# Autodesk Inventor assembly: ASY GBK 3310 central wall shield 7
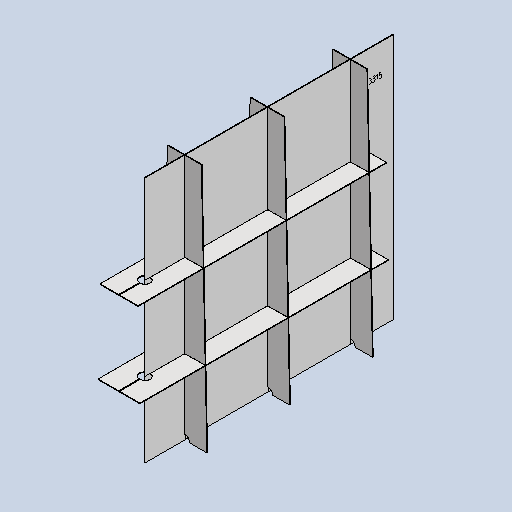
[picture p0: Inventor's stored thumbnail of the model, 512x512]
Saved by Autodesk Inventor 2026.2 (Build 302298010, 298A)
## iProperties
Created: 2026-05-19
Part Number: ASY GBK 3310 central wall shield 7
Document SubType Name: Assembly
Designer: pokla
Mass: 123029 g
Surface Area: 79995.2 cm^2
Volume: 15672.5 cm^3
Density: 7.85 g/cm^3
Author: admin
## Documents named in this file (6)
- C:\Users\admin\Documents\Inventor\GBK-Gubkinskiy\ASY GBK 3310 central wall shield 7.iam
- C:\Users\admin\Documents\Inventor\GBK-Gubkinskiy\GBK 3312 stringer 7.ipt
- C:\Users\admin\Documents\Inventor\GBK-Gubkinskiy\GBK 3317 shield 7.ipt
- C:\Users\admin\Documents\Inventor\GBK-Gubkinskiy\GBK 3313 stringer 8.ipt
- C:\Users\admin\Documents\Inventor\GBK-Gubkinskiy\GBK 3311 central third rib.ipt
- C:\Users\admin\Documents\Inventor\GBK-Gubkinskiy\GBK 0101 main rib.ipt
## Components (11 placed, 4 different names)
1. GBK 3312 stringer 7.ipt:1 — Rigid:1
2. GBK 3317 shield 7.ipt:1 — Flush:7, Flush:5, Mate:5, Mate:2, Flush:1, Mate:1, Flush:6, Mate:4
3. GBK 3313 stringer 8.ipt:1 — Rigid:2
4. GBK 3312 stringer 7.ipt:2 — Rigid:4
5. GBK 3313 stringer 8.ipt:2 — Rigid:3
6. GBK 3311 central third rib.ipt:1 — Flush:6, Flush:4, Mate:4, Rigid:4, Rigid:3
7. GBK 3311 central third rib.ipt:2 — Flush:7, Flush:5, Mate:5, Flush:4, Rigid:1, Rigid:2
8. GBK 3311 central third rib.ipt:3
9. GBK 3311 central third rib.ipt:4
10. GBK 3311 central third rib.ipt:5
11. GBK 3311 central third rib.ipt:6
## Component patterns: (3 elements, first: GBK 3311 central third rib.ipt:1 + GBK 3311 central third rib.ipt:2)
## Relationships (13: Flush 5, Mate 4, WeldJoint 4)
- Flush:7: GBK 3317 shield 7.ipt:1 ↔ GBK 3311 central third rib.ipt:2
- Flush:5 (254 mm): GBK 3317 shield 7.ipt:1 ↔ GBK 3311 central third rib.ipt:2
- Mate:5: GBK 3317 shield 7.ipt:1 ↔ GBK 3311 central third rib.ipt:2
- Mate:2: GBK 3317 shield 7.ipt:1
- Flush:1: GBK 3317 shield 7.ipt:1
- Mate:1: GBK 3317 shield 7.ipt:1
- Flush:6: GBK 3317 shield 7.ipt:1 ↔ GBK 3311 central third rib.ipt:1
- Flush:4: GBK 3311 central third rib.ipt:1 ↔ GBK 3311 central third rib.ipt:2
- Mate:4: GBK 3317 shield 7.ipt:1 ↔ GBK 3311 central third rib.ipt:1
- Rigid:1 [WeldJoint] (4 mm): GBK 3312 stringer 7.ipt:1 ↔ GBK 3311 central third rib.ipt:2
- Rigid:2 [WeldJoint] (4 mm): GBK 3313 stringer 8.ipt:1 ↔ GBK 3311 central third rib.ipt:2
- Rigid:4 [WeldJoint] (4 mm): GBK 3312 stringer 7.ipt:2 ↔ GBK 3311 central third rib.ipt:1
- Rigid:3 [WeldJoint] (4 mm): GBK 3313 stringer 8.ipt:2 ↔ GBK 3311 central third rib.ipt:1
## Named parameters: Шаг_шпангоутов = 496.66667 mm
